# Autodesk Inventor assembly: Assembly1
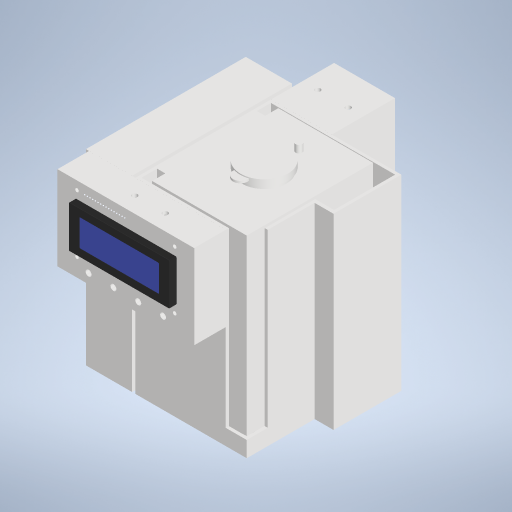
[picture p0: Inventor's stored thumbnail of the model, 512x512]
Saved by Autodesk Inventor 2023 (Build 270158030, 158C)
## iProperties
Created: 2023-03-05
Part Number: Assembly1
Document SubType Name: Assembly
Designer: fatih
Author: fatih
## Documents named in this file (8)
- C:\Users\fatih\Documents\Inventor\Pengmas Hidroponik\Assembly1.iam
- C:\Users\fatih\Documents\Inventor\Pengmas Hidroponik\cover windshield.ipt
- C:\Users\fatih\Documents\Inventor\Pengmas Hidroponik\windshield washer.ipt
- C:\Users\fatih\Documents\Inventor\Pengmas Hidroponik\port side.ipt
- C:\Users\fatih\Documents\Inventor\Pengmas Hidroponik\port plugin.ipt
- C:\Users\fatih\Documents\Inventor\Pengmas Hidroponik\lcd-20x4-i2c-1.snapshot.4\Lcd i2c.ipt
- C:\Users\fatih\Documents\Inventor\Pengmas Hidroponik\cover lcd.ipt
- C:\Users\fatih\Documents\Inventor\Pengmas Hidroponik\back side.ipt
## Components (7 placed, 7 different names)
1. cover windshield:1 — Mate:1, Mate:2, Flush:1, Flush:2, Mate:6, Flush:3, Flush:4, Mate:10, Mate:12
2. windshield washer:1 — Mate:1, Mate:2
3. port side:1 — Flush:1, Flush:2, Mate:3, Mate:4, Mate:5, Mate:6
4. port plugin:1 — Mate:3, Mate:4, Mate:5
5. Lcd i2c:1 — Mate:7, Mate:8, Mate:9
6. cover lcd:1 — Mate:7, Mate:8, Mate:9, Flush:3, Flush:4, Mate:10, Mate:11, Flush:5
7. back side:1 — Mate:11, Flush:5, Mate:12
## Relationships (17: Mate 12, Flush 5)
- Mate:1: cover windshield:1 ↔ windshield washer:1
- Mate:2: cover windshield:1 ↔ windshield washer:1
- Flush:1: cover windshield:1 ↔ port side:1
- Flush:2: cover windshield:1 ↔ port side:1
- Mate:3: port side:1 ↔ port plugin:1
- Mate:4: port side:1 ↔ port plugin:1
- Mate:5: port side:1 ↔ port plugin:1
- Mate:6: cover windshield:1 ↔ port side:1
- Mate:7: Lcd i2c:1 ↔ cover lcd:1
- Mate:8: Lcd i2c:1 ↔ cover lcd:1
- Mate:9: Lcd i2c:1 ↔ cover lcd:1
- Flush:3: cover windshield:1 ↔ cover lcd:1
- Flush:4: cover windshield:1 ↔ cover lcd:1
- Mate:10: cover windshield:1 ↔ cover lcd:1
- Mate:11: cover lcd:1 ↔ back side:1
- Flush:5: cover lcd:1 ↔ back side:1
- Mate:12: cover windshield:1 ↔ back side:1
